# Autodesk Inventor assembly: base
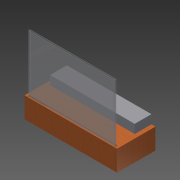
[picture p0: Inventor's stored thumbnail of the model, 180x180]
Saved by Autodesk Inventor 2013 (Build 170138000, 138)
## iProperties
Created: 2013-05-01
Part Number: base
Document SubType Name: Assembly
Designer: Chris
Mass: 92224.3 g
Surface Area: 146571 cm^2
Volume: 108180 cm^3
Density: 0.852507 g/cm^3
Author: Chris
## Documents named in this file (10)
- C:\Users\Chris\Documents\Inventor\Redbull-2013\base-v1\base.iam
- C:\Users\Chris\Documents\Inventor\Redbull-2013\base-v1\bottom-plate.ipt
- C:\Users\Chris\Documents\Inventor\Redbull-2013\base-v1\front-plate.ipt
- C:\Users\Chris\Documents\Inventor\Redbull-2013\base-v1\top-plate.ipt
- C:\Users\Chris\Documents\Inventor\Redbull-2013\bubble-wall-final\bubble-wall.iam
- C:\Users\Chris\Documents\Inventor\Redbull-2013\base-v1\side.ipt
- C:\Users\Chris\Documents\Inventor\Redbull-2013\base-v1\tank-guide.ipt
- C:\Users\Chris\Documents\Inventor\Redbull-2013\base-v1\bottom-guide.ipt
- C:\Users\Chris\Documents\Inventor\Redbull-2013\base-v1\back-plate.ipt
- C:\Users\Chris\Documents\Inventor\Redbull-2013\piano-placeholder.ipt
## Components (11 placed, 9 different names)
1. bottom-plate:1 — Mate:1, Flush:1, Flush:2, Flush:3, Mate:2, Flush:4, Mate:4, Flush:7, Mate:8, Mate:9, Flush:10, Mate:16
2. front-plate:1 — Mate:1, Flush:1, Flush:2, Mate:3, Flush:5
3. back-plate:1 — Flush:3, Mate:2, Flush:4, Flush:6, Mate:7, Mate:11, Flush:13
4. top-plate:1 — Mate:3, Flush:5, Flush:6, Mate:5, Mate:6, Mate:19
5. bubble-wall:1 [sub-assembly] — Mate:4, Mate:5, Mate:6, Mate:14, Mate:15, Mate:18
6. side:1 — Flush:7, Mate:7, Mate:8, Mate:12, Flush:11
7. side:2 — Mate:9, Flush:10, Mate:11, Mate:13, Flush:12, Mate:17, Flush:14
8. tank-guide:1 — Mate:12, Flush:11, Mate:15
9. tank-guide:2 — Mate:13, Flush:12, Mate:14
10. bottom-guide:1 — Mate:16, Mate:17, Mate:18
11. piano-placeholder:1 — Mate:19, Flush:13, Flush:14
## Relationships (30: Mate 18, Flush 12)
- Mate:1: bottom-plate:1 ↔ front-plate:1
- Flush:1: bottom-plate:1 ↔ front-plate:1
- Flush:2: bottom-plate:1 ↔ front-plate:1
- Flush:3: bottom-plate:1 ↔ back-plate:1
- Mate:2: bottom-plate:1 ↔ back-plate:1
- Flush:4: bottom-plate:1 ↔ back-plate:1
- Mate:3: front-plate:1 ↔ top-plate:1
- Flush:5: front-plate:1 ↔ top-plate:1
- Flush:6: back-plate:1 ↔ top-plate:1
- Mate:4: bottom-plate:1 ↔ bubble-wall:1
- Mate:5: top-plate:1 ↔ bubble-wall:1
- Mate:6: top-plate:1 ↔ bubble-wall:1
- Flush:7: bottom-plate:1 ↔ side:1
- Mate:7: back-plate:1 ↔ side:1
- Mate:8: bottom-plate:1 ↔ side:1
- Mate:9: bottom-plate:1 ↔ side:2
- Flush:10: bottom-plate:1 ↔ side:2
- Mate:11: back-plate:1 ↔ side:2
- Mate:12: side:1 ↔ tank-guide:1
- Flush:11: side:1 ↔ tank-guide:1
- Mate:13: side:2 ↔ tank-guide:2
- Flush:12: side:2 ↔ tank-guide:2
- Mate:14: bubble-wall:1 ↔ tank-guide:2
- Mate:15: bubble-wall:1 ↔ tank-guide:1
- Mate:16: bottom-plate:1 ↔ bottom-guide:1
- Mate:17: side:2 ↔ bottom-guide:1
- Mate:18: bubble-wall:1 ↔ bottom-guide:1
- Mate:19: top-plate:1 ↔ piano-placeholder:1
- Flush:13: back-plate:1 ↔ piano-placeholder:1
- Flush:14 (63.5 mm): side:2 ↔ piano-placeholder:1
